# Autodesk Inventor assembly: Shoulder_nema23
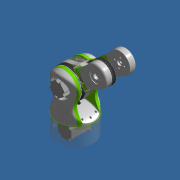
[picture p0: Inventor's stored thumbnail of the model, 180x180]
Saved by Autodesk Inventor 2016 (Build 200138000, 138)
## iProperties
Created: 2015-01-06
Part Number: Shoulder_nema23
Document SubType Name: Assembly
Designer: 4ndreas
Author: 4ndreas
## Documents named in this file (16)
- C:\Users\4ndreas\Documents\Inventor\RobotARM v2\v4\Shoulder_nema23.iam
- C:\Users\4ndreas\Documents\Inventor\RobotARM v2\v2\BaseJoint\Konstruktions-Assistent\Übertragung des Zahnriemens1.iam
- C:\Users\4ndreas\Documents\Inventor\Content Center Files\R2014\de-DE\DIN 125-1  A\DIN 125 - A 4,3.ipt
- C:\Users\4ndreas\Documents\Inventor\Content Center Files\R2014\de-DE\DIN BEARING(1)\DIN 625 SKF - SKF 624.ipt
- C:\Users\4ndreas\Documents\Inventor\Content Center Files\R2014\de-DE\DIN 433-1  A\DIN 433 - 4,3.ipt
- C:\Users\4ndreas\Documents\Inventor\RobotARM v2\v3\Shouder_spanner_Scheibe.ipt
- C:\Users\4ndreas\Documents\Inventor\RobotARM v2\v3\Shoulder_spanner.ipt
- C:\Users\4ndreas\Documents\Inventor\Content Center Files\R2014\de-DE\DIN 934\DIN 934 - M4 x 0,7.ipt
- C:\Users\4ndreas\Documents\Inventor\RobotARM v2\v2\encoder.iam
- C:\Users\4ndreas\Documents\Inventor\Content Center Files\R2014\de-DE\DIN 912\DIN 912 - M4 x 0,7 x 35 x 20.ipt
- C:\Users\4ndreas\Documents\Inventor\RobotARM v2\v4\Shoulder_stepper\Konstruktions-Assistent\Übertragung des Zahnriemens1.iam
- C:\Users\4ndreas\Documents\Inventor\RobotARM v2\v4\Ellbow.iam
- C:\Users\4ndreas\Documents\Inventor\RobotARM v2\v4\Nema24.ipt
- C:\Users\4ndreas\Documents\Inventor\Content Center Files\R2014\de-DE\DIN BEARING(1)\DIN 625 SKF - SKF 61818.ipt
- C:\Users\4ndreas\Documents\Inventor\RobotARM v2\v4\Shoulder_basis_N24.ipt
- C:\Users\4ndreas\Documents\Inventor\RobotARM v2\v4\CoverBase.ipt
## Components (26 placed, 14 different names)
1. Übertragung des Zahnriemens:1 [sub-assembly] — Passend:1, Passend:12, Passend:49, Passend:69, Passend:72, Passend:94, Passend:95, Passend:137, Passend:138
2. DIN 912 - ersetzt durch DIN EN ISO 4762 M4 x 35:2 — Passend:70, Passend:71, Passend:72, Passend:77, Passend:78, Passend:87, Passend:88, Passend:91, Passend:97
3. DIN 912 - ersetzt durch DIN EN ISO 4762 M4 x 35:1 — Passend:69, Passend:73, Passend:74, Passend:82, Passend:83, Passend:85, Passend:99, Passend:104
4. DIN 125-1 A A 4,3:1 — Passend:70, Passend:71, Fluchtend:9
5. DIN 125-1 A A 4,3:2 — Passend:73, Passend:74, Fluchtend:9
6. DIN 625 SKF 624:1 — Passend:78, Passend:79, Passend:90
7. DIN 625 SKF 624:2 — Passend:77, Passend:79, Passend:89
8. DIN 625 SKF 624:3 — Passend:80, Passend:81, Passend:82, Passend:84
9. DIN 625 SKF 624:4 — Passend:80, Passend:81, Passend:86
10. DIN 433-1 A 4,3:1 — Passend:87, Passend:90, Passend:103
11. DIN 433-1 A 4,3:2 — Passend:83, Passend:84
12. DIN 433-1 A 4,3:3 — Passend:85, Passend:86, Passend:105
13. DIN 433-1 A 4,3:4 — Passend:88, Passend:89
14. Shoulder_spanner:1 — Passend:94, Passend:95, Passend:96, Passend:98, Passend:100, Passend:101, Passend:102
15. Shouder_spanner_Scheibe:2 — Passend:91, Passend:103
16. DIN 934 - ersetzt durch DIN EN 24032/28673/28674 M4:1 — Passend:99, Passend:100, Passend:101
17. DIN 934 - ersetzt durch DIN EN 24032/28673/28674 M4:2 — Passend:97, Passend:98, Passend:102
18. Shouder_spanner_Scheibe:3 — Passend:104, Passend:105
19. encoder:2 [sub-assembly] — Passend:116
20. Übertragung des Zahnriemens:2 [sub-assembly] — Passend:130, Passend:131
21. Nema24:1 — Passend:130, Passend:131, Winkel:10
22. Ellbow:1 [sub-assembly] — Passend:137, Passend:141
23. DIN 625 SKF SKF 61818:1 — Passend:138, Passend:141, Passend:142
24. Shoulder_basis_N24:1 — Passend:139, Fluchtend:14, Passend:140, Fluchtend:16, Passend:142, Passend:143, Passend:144, Fluchtend:17
25. CoverBase:1 — Passend:143
26. DIN 625 SKF SKF 61818:2 — Passend:144, Fluchtend:17
## Relationships (57: Mate 50, Flush 6, Angle 1)
- Passend:1 [Mate]: Übertragung des Zahnriemens:1
- Passend:4 [Mate]
- Passend:12 [Mate]: Übertragung des Zahnriemens:1
- Passend:49 [Mate]: Übertragung des Zahnriemens:1
- Passend:62 [Mate]
- Passend:63 [Mate]
- Passend:69 [Mate]: Übertragung des Zahnriemens:1 ↔ DIN 912 - ersetzt durch DIN EN ISO 4762 M4 x 35:1
- Passend:70 [Mate]: DIN 912 - ersetzt durch DIN EN ISO 4762 M4 x 35:2 ↔ DIN 125-1 A A 4,3:1
- Passend:71 [Mate]: DIN 912 - ersetzt durch DIN EN ISO 4762 M4 x 35:2 ↔ DIN 125-1 A A 4,3:1
- Passend:72 [Mate]: Übertragung des Zahnriemens:1 ↔ DIN 912 - ersetzt durch DIN EN ISO 4762 M4 x 35:2
- Passend:73 [Mate]: DIN 912 - ersetzt durch DIN EN ISO 4762 M4 x 35:1 ↔ DIN 125-1 A A 4,3:2
- Passend:74 [Mate]: DIN 912 - ersetzt durch DIN EN ISO 4762 M4 x 35:1 ↔ DIN 125-1 A A 4,3:2
- Passend:77 [Mate]: DIN 912 - ersetzt durch DIN EN ISO 4762 M4 x 35:2 ↔ DIN 625 SKF 624:2
- Passend:78 [Mate]: DIN 912 - ersetzt durch DIN EN ISO 4762 M4 x 35:2 ↔ DIN 625 SKF 624:1
- Passend:79 [Mate]: DIN 625 SKF 624:1 ↔ DIN 625 SKF 624:2
- Passend:80 [Mate]: DIN 625 SKF 624:3 ↔ DIN 625 SKF 624:4
- Passend:81 [Mate]: DIN 625 SKF 624:3 ↔ DIN 625 SKF 624:4
- Passend:82 [Mate]: DIN 912 - ersetzt durch DIN EN ISO 4762 M4 x 35:1 ↔ DIN 625 SKF 624:3
- Passend:83 [Mate]: DIN 912 - ersetzt durch DIN EN ISO 4762 M4 x 35:1 ↔ DIN 433-1 A 4,3:2
- Passend:84 [Mate]: DIN 625 SKF 624:3 ↔ DIN 433-1 A 4,3:2
- Passend:85 [Mate]: DIN 912 - ersetzt durch DIN EN ISO 4762 M4 x 35:1 ↔ DIN 433-1 A 4,3:3
- Passend:86 [Mate]: DIN 625 SKF 624:4 ↔ DIN 433-1 A 4,3:3
- Passend:87 [Mate]: DIN 912 - ersetzt durch DIN EN ISO 4762 M4 x 35:2 ↔ DIN 433-1 A 4,3:1
- Passend:88 [Mate]: DIN 912 - ersetzt durch DIN EN ISO 4762 M4 x 35:2 ↔ DIN 433-1 A 4,3:4
- Passend:89 [Mate]: DIN 625 SKF 624:2 ↔ DIN 433-1 A 4,3:4
- Passend:90 [Mate]: DIN 625 SKF 624:1 ↔ DIN 433-1 A 4,3:1
- Passend:91 [Mate]: DIN 912 - ersetzt durch DIN EN ISO 4762 M4 x 35:2 ↔ Shouder_spanner_Scheibe:2
- Passend:94 [Mate]: Übertragung des Zahnriemens:1 ↔ Shoulder_spanner:1
- Passend:95 [Mate]: Übertragung des Zahnriemens:1 ↔ Shoulder_spanner:1
- Passend:96 [Mate]: Shoulder_spanner:1
- Passend:97 [Mate]: DIN 912 - ersetzt durch DIN EN ISO 4762 M4 x 35:2 ↔ DIN 934 - ersetzt durch DIN EN 24032/28673/28674 M4:2
- Passend:98 [Mate]: Shoulder_spanner:1 ↔ DIN 934 - ersetzt durch DIN EN 24032/28673/28674 M4:2
- Passend:99 [Mate]: DIN 912 - ersetzt durch DIN EN ISO 4762 M4 x 35:1 ↔ DIN 934 - ersetzt durch DIN EN 24032/28673/28674 M4:1
- Passend:100 [Mate]: Shoulder_spanner:1 ↔ DIN 934 - ersetzt durch DIN EN 24032/28673/28674 M4:1
- Passend:101 [Mate]: Shoulder_spanner:1 ↔ DIN 934 - ersetzt durch DIN EN 24032/28673/28674 M4:1
- Passend:102 [Mate]: Shoulder_spanner:1 ↔ DIN 934 - ersetzt durch DIN EN 24032/28673/28674 M4:2
- Passend:103 [Mate]: DIN 433-1 A 4,3:1 ↔ Shouder_spanner_Scheibe:2
- Passend:104 [Mate]: DIN 912 - ersetzt durch DIN EN ISO 4762 M4 x 35:1 ↔ Shouder_spanner_Scheibe:3
- Passend:105 [Mate]: DIN 433-1 A 4,3:3 ↔ Shouder_spanner_Scheibe:3
- Fluchtend:9 [Flush]: DIN 125-1 A A 4,3:1 ↔ DIN 125-1 A A 4,3:2
- Passend:116 [Mate]: encoder:2
- Fluchtend:12 [Flush] (43 mm)
- Fluchtend:13 [Flush] (20 mm)
- Passend:130 [Mate]: Übertragung des Zahnriemens:2 ↔ Nema24:1
- Passend:131 [Mate] (3 mm): Übertragung des Zahnriemens:2 ↔ Nema24:1
- Winkel:10 [Angle] (0 deg): Nema24:1
- Passend:137 [Mate]: Übertragung des Zahnriemens:1 ↔ Ellbow:1
- Passend:138 [Mate]: Übertragung des Zahnriemens:1 ↔ DIN 625 SKF SKF 61818:1
- Passend:139 [Mate]: Shoulder_basis_N24:1
- Fluchtend:14 [Flush]: Shoulder_basis_N24:1
- Passend:140 [Mate]: Shoulder_basis_N24:1
- Fluchtend:16 [Flush]: Shoulder_basis_N24:1
- Passend:141 [Mate]: Ellbow:1 ↔ DIN 625 SKF SKF 61818:1
- Passend:142 [Mate]: DIN 625 SKF SKF 61818:1 ↔ Shoulder_basis_N24:1
- Passend:143 [Mate]: Shoulder_basis_N24:1 ↔ CoverBase:1
- Passend:144 [Mate]: Shoulder_basis_N24:1 ↔ DIN 625 SKF SKF 61818:2
- Fluchtend:17 [Flush]: Shoulder_basis_N24:1 ↔ DIN 625 SKF SKF 61818:2
